# Autodesk Inventor assembly: 1x2Pins
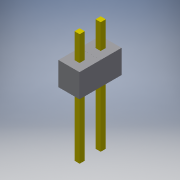
[picture p0: Inventor's stored thumbnail of the model, 180x180]
Saved by Autodesk Inventor 2019 (Build 230136000, 136)
## iProperties
Created: 2019-07-16
Part Number: 1x2Pins
Document SubType Name: Assembly
Designer: james
Author: james
## Documents named in this file (2)
- F:\JimsDesign\P1001-16bit-CPU\P1001-001 - 16bit CPU\P1001-001-210 - CAD Library\1x2Pins.iam
- F:\JimsDesign\P1001-16bit-CPU\P1001-001 - 16bit CPU\P1001-001-210 - CAD Library\1FullPin.iam
## Components (2 placed, 1 different names)
1. 1FullPin:1 [sub-assembly] — Mate:1, Flush:1, Flush:2
2. 1FullPin:2 [sub-assembly] — Mate:1, Flush:1, Flush:2
## Relationships (3: Flush 2, Mate 1)
- Mate:1: 1FullPin:1 ↔ 1FullPin:2
- Flush:1: 1FullPin:1 ↔ 1FullPin:2
- Flush:2: 1FullPin:1 ↔ 1FullPin:2
